# Autodesk Inventor assembly: Mecanismo
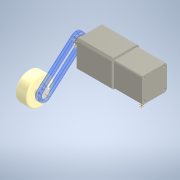
[picture p0: Inventor's stored thumbnail of the model, 180x180]
Saved by Autodesk Inventor 2022.1 (Build 261234000, 234)
## iProperties
Created: 2021-09-11
Part Number: Mecanismo
Document SubType Name: Assembly
Designer: seb_0
Author: seb_0
## Documents named in this file (6)
- C:\Users\seb_0\Desktop\RobotPallet_v2\Mecanismo de movimiento\Mecanismo - Derecho.iam
- C:\Users\seb_0\Desktop\RobotPallet_v2\Mecanismo de movimiento\Rueda.ipt
- C:\Users\seb_0\Desktop\RobotPallet_v2\Mecanismo de movimiento\Eje.ipt
- C:\Users\seb_0\Desktop\RobotPallet_v2\Mecanismo de movimiento\Motor 1KW.ipt
- C:\Users\seb_0\Desktop\RobotPallet_v2\Mecanismo de movimiento\Caja reductora 1KW.ipt
- C:\Users\seb_0\Desktop\RobotPallet_v2\Mecanismo de movimiento\Mecanismo - Derecho\Design Accelerator\Transmisión por cadena1.iam
## Components (5 placed, 5 different names)
1. Rueda:1 — Nivelación:1, Coincidencia:7, Coincidencia:9
2. Eje:1 — Nivelación:1, Coincidencia:7, Coincidencia:8
3. Motor 1KW:1 — Coincidencia:2, Coincidencia:3, Coincidencia:4, Coincidencia:5, Coincidencia:6, Nivelación:2
4. Caja reductora 1KW:1 — Coincidencia:2, Coincidencia:3, Nivelación:2
5. Transmisión por cadena:1 [sub-assembly] — Coincidencia:8, Coincidencia:9
## Relationships (10: Mate 8, Flush 2)
- Nivelación:1 [Flush]: Rueda:1 ↔ Eje:1
- Coincidencia:2 [Mate]: Motor 1KW:1 ↔ Caja reductora 1KW:1
- Coincidencia:3 [Mate] (5 mm): Motor 1KW:1 ↔ Caja reductora 1KW:1
- Coincidencia:4 [Mate]: Motor 1KW:1
- Coincidencia:5 [Mate] (9.5 mm): Motor 1KW:1
- Coincidencia:6 [Mate]: Motor 1KW:1
- Coincidencia:7 [Mate]: Rueda:1 ↔ Eje:1
- Nivelación:2 [Flush] (5 mm): Motor 1KW:1 ↔ Caja reductora 1KW:1
- Coincidencia:8 [Mate]: Eje:1 ↔ Transmisión por cadena:1
- Coincidencia:9 [Mate] (10 mm): Rueda:1 ↔ Transmisión por cadena:1
